# Autodesk Inventor assembly: Assembly_Lasergroup_wPickup
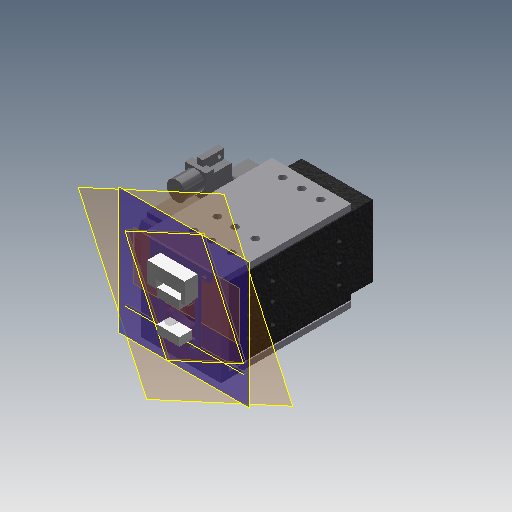
[picture p0: Inventor's stored thumbnail of the model, 512x512]
Saved by Autodesk Inventor 2019 (Build 230136000, 136)
## iProperties
Created: 2019-04-21
Part Number: Assembly_Lasergroup_wPickup
Document SubType Name: Assembly
Designer: diederichbenedict
Author: diederichbenedict
## Documents named in this file (5)
- C:\Users\diederichbenedict\Dropbox\Dokumente\Promotion\PROJECTS\STORMoChip\INVENTOR\Nanoscopy-on-a-cheap\Assembly_Lasergroup_wPickup.iam
- C:\Users\diederichbenedict\Dropbox\Dokumente\Promotion\PROJECTS\STORMoChip\INVENTOR\Nanoscopy-on-a-cheap\00_LASER_640nm.ipt
- C:\Users\diederichbenedict\Dropbox\Dokumente\Promotion\PROJECTS\STORMoChip\INVENTOR\Nanoscopy-on-a-cheap\01_XY_Actuator.ipt
- C:\Users\diederichbenedict\Dropbox\Dokumente\Promotion\PROJECTS\STORMoChip\INVENTOR\Nanoscopy-on-a-cheap\10_Adapterplate_Laser.ipt
- C:\Users\diederichbenedict\Dropbox\Dokumente\Promotion\PROJECTS\STORMoChip\INVENTOR\Nanoscopy-on-a-cheap\00_KES400.iam
## Components (4 placed, 4 different names)
1. 00_LASER_640nm:1 — Mate:2
2. 01_XY_Actuator:1 — Flush:3, Flush:4
3. 10_Adapterplate_Laser:1 — Flush:3, Flush:4, Angle:1, Mate:3
4. 00_KES400:1 [sub-assembly] — Mate:2, Angle:1, Mate:3
## Relationships (8: Flush 4, Mate 3, Angle 1)
- [Mate] (7 mm): 00_LASER_640nm:1 ↔ 01_XY_Actuator:1
- [Flush]: 00_LASER_640nm:1 ↔ 01_XY_Actuator:1
- [Flush]: 00_LASER_640nm:1 ↔ 01_XY_Actuator:1
- Flush:3: 01_XY_Actuator:1 ↔ 10_Adapterplate_Laser:1
- Flush:4: 01_XY_Actuator:1 ↔ 10_Adapterplate_Laser:1
- Mate:2: 00_LASER_640nm:1 ↔ 00_KES400:1
- Angle:1 (180 deg): 10_Adapterplate_Laser:1 ↔ 00_KES400:1
- Mate:3: 10_Adapterplate_Laser:1 ↔ 00_KES400:1
